# Autodesk Inventor assembly: 3 Motor Gearbox
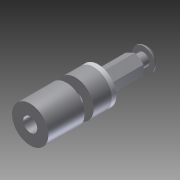
[picture p0: Inventor's stored thumbnail of the model, 180x180]
Saved by Autodesk Inventor 2014 SP1 (Build 180222100, 222)
## iProperties
Created: 2013-10-10
Part Number: 3 Motor Gearbox
Document SubType Name: Assembly
Designer: RyanHughes
Author: Andrew
Title: E:\My Documents\Inventor\VEX Robots\Sack Attack\15 defense\3 Motor Gearbox.stp
Creation Date: 2013-01-16
Sending System: Autodesk Inventor 2013
Preprocessor: Autodesk Inventor 2013
Author: RyanHughes
## Documents named in this file (6)
- C:\Users\Ryan\Desktop\sw\toss up 2ed A bot\drivetrain\spacer for gearbox.iam
- C:\Users\Ryan\Desktop\sw\lib\Aperture VEX CAD Library\Spacers\SPACER-0500-0500.ipt
- C:\Users\Ryan\Desktop\sw\lib\Aperture VEX CAD Library\Spacers\SPACER-0500-0625.ipt
- C:\Users\Ryan\Desktop\sw\lib\Aperture VEX CAD Library\Standoffs\BEAM-0500.ipt
- C:\Users\Ryan\Desktop\sw\lib\Aperture VEX CAD Library\Spacers\SPACER-0500-0250.ipt
- C:\Users\Ryan\Desktop\sw\lib\Aperture VEX CAD Library\Hardware\8-32\8-32_.250.ipt
## Components (5 placed, 5 different names)
1. SPACER-0500-0500:3 — Mate:39, Mate:40
2. BEAM-0500:3 — Mate:35, Mate:38, Mate:42
3. SPACER-0500-0250:1 — Mate:35, Mate:36, Mate:37, Mate:39, Mate:40, Mate:41
4. SPACER-0500-0625:1 — Mate:36, Mate:37, Mate:38
5. 8-32_.250:1 — Mate:41, Mate:42
## Relationships (8: Mate 8)
- Mate:35: BEAM-0500:3 ↔ SPACER-0500-0250:1
- Mate:36: SPACER-0500-0250:1 ↔ SPACER-0500-0625:1
- Mate:37: SPACER-0500-0250:1 ↔ SPACER-0500-0625:1
- Mate:38: BEAM-0500:3 ↔ SPACER-0500-0625:1
- Mate:39 (3.175 mm): SPACER-0500-0500:3 ↔ SPACER-0500-0250:1
- Mate:40: SPACER-0500-0500:3 ↔ SPACER-0500-0250:1
- Mate:41: SPACER-0500-0250:1 ↔ 8-32_.250:1
- Mate:42 (3.175 mm): BEAM-0500:3 ↔ 8-32_.250:1
